# Autodesk Inventor assembly: BV-ASM-222-106
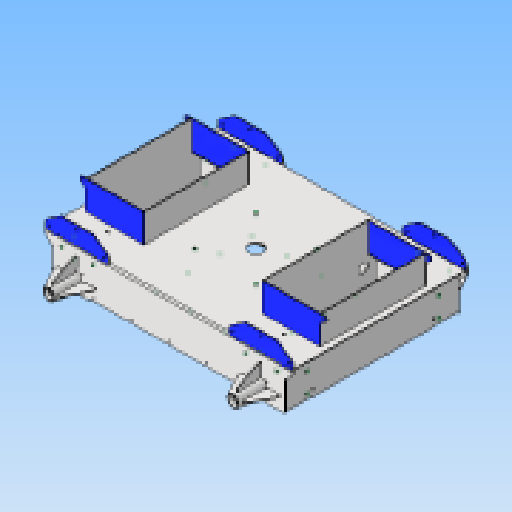
[picture p0: Inventor's stored thumbnail of the model, 512x512]
Saved by Autodesk Inventor 2025.4 (Build 294407000, 407)
## iProperties
Created: 2025-12-05
Part Number: BV-ASM-222-106
Document SubType Name: Assembly
Designer: josh
Mass: 150690 g
Surface Area: 81440.8 cm^2
Volume: 19196.2 cm^3
Density: 7.85 g/cm^3
Description: Base Weldment
Author: josh
## iProperties of the stored document MemberDocs/x54frrunuJ0si20qmEdadrqylTg
Created: 2025-12-05
Document SubType Name: Assembly
Designer: josh
Mass: 150690 g
Surface Area: 81440.8 cm^2
Volume: 19196.2 cm^3
Density: 7.85 g/cm^3
Author: josh
## iProperties of the stored document MemberDocs/xFojfi5agHc25u2sk4sonpsnbLc
Created: 2025-12-05
Document SubType Name: Assembly
Designer: josh
Mass: 150690 g
Surface Area: 81440.8 cm^2
Volume: 19196.2 cm^3
Density: 7.85 g/cm^3
Author: josh
## Documents named in this file (30)
- R:\A1- Neuweg Design Data\OM Robotics\BASE VEHICLE DESIGN PROJECT\BV-ASM-222-106.iam
- R:\A1- Neuweg Design Data\OM Robotics\BASE VEHICLE DESIGN PROJECT\BV-222-106.ipt
- R:\A1- Neuweg Design Data\OM Robotics\BASE VEHICLE DESIGN PROJECT\BV-222-107.ipt
- R:\A1- Neuweg Design Data\OM Robotics\BASE VEHICLE DESIGN PROJECT\BV-222-109.ipt
- R:\A1- Neuweg Design Data\OM Robotics\BASE VEHICLE DESIGN PROJECT\BV-222-116.ipt
- R:\A1- Neuweg Design Data\OM Robotics\BASE VEHICLE DESIGN PROJECT\BV-222-117.ipt
- R:\A1- Neuweg Design Data\OM Robotics\BASE VEHICLE DESIGN PROJECT\BV-222-118.ipt
- R:\A1- Neuweg Design Data\OM Robotics\BASE VEHICLE DESIGN PROJECT\BV-ASM-222-104.iam
- R:\A1- Neuweg Design Data\OM Robotics\BASE VEHICLE DESIGN PROJECT\BV-ASM-222-105.iam
- R:\A1- Neuweg Design Data\OM Robotics\BASE VEHICLE DESIGN PROJECT\BV-222-105.ipt
- R:\A1- Neuweg Design Data\OM Robotics\BASE VEHICLE DESIGN PROJECT\BV-222-108.ipt
- R:\A1- Neuweg Design Data\OM Robotics\BASE VEHICLE DESIGN PROJECT\BV-222-112.ipt
- R:\A1- Neuweg Design Data\OM Robotics\BASE VEHICLE DESIGN PROJECT\BV-222-119.ipt
- R:\A1- Neuweg Design Data\OM Robotics\BASE VEHICLE DESIGN PROJECT\BV-222-120.ipt
- R:\A1- Neuweg Design Data\OM Robotics\BASE VEHICLE DESIGN PROJECT\0222-110.ipt
- R:\A1- Neuweg Design Data\OM Robotics\BASE VEHICLE DESIGN PROJECT\3_8-16 x 5_8 Flange Bolt.ipt
- R:\A1- Neuweg Design Data\OM Robotics\BASE VEHICLE DESIGN PROJECT\1_4-20 UNC x 0.625.ipt
- R:\A1- Neuweg Design Data\OM Robotics\BASE VEHICLE DESIGN PROJECT\90128A277.ipt
- R:\A1- Neuweg Design Data\OM Robotics\BASE VEHICLE DESIGN PROJECT\91290A446.ipt
- R:\A1- Neuweg Design Data\OM Robotics\BASE VEHICLE DESIGN PROJECT\91259A177.ipt
- R:\A1- Neuweg Design Data\OM Robotics\BASE VEHICLE DESIGN PROJECT\94945A213.ipt
- R:\A1- Neuweg Design Data\OM Robotics\BASE VEHICLE DESIGN PROJECT\BV-ASM-222-102.iam
- R:\A1- Neuweg Design Data\OM Robotics\BASE VEHICLE DESIGN PROJECT\30205.ipt
- R:\A1- Neuweg Design Data\OM Robotics\BASE VEHICLE DESIGN PROJECT\251105 Motor_Drive.ipt
- R:\A1- Neuweg Design Data\OM Robotics\BASE VEHICLE DESIGN PROJECT\22x10x8.ipt
- R:\A1- Neuweg Design Data\OM Robotics\BASE VEHICLE DESIGN PROJECT\0222-113-2.ipt
- R:\A1- Neuweg Design Data\OM Robotics\BASE VEHICLE DESIGN PROJECT\97260A109.ipt
- R:\A1- Neuweg Design Data\OM Robotics\BASE VEHICLE DESIGN PROJECT\93560A112.ipt
- R:\A1- Neuweg Design Data\OM Robotics\BASE VEHICLE DESIGN PROJECT\1199N323.ipt
- R:\A1- Neuweg Design Data\OM Robotics\BASE VEHICLE DESIGN PROJECT\BV-ASM-222-103.iam
## Components (30 placed, 8 different names)
1. BV-ASM-222-104:1 [sub-assembly] — Flush:11, Flush:12, Flush:13
2. BV-ASM-222-105:1 [sub-assembly]
3. BV-222-106:1
4. BV-222-107:1
5. BV-222-109:1
6. BV-222-116:1
7. BV-222-118:1
8. BV-222-106:2
9. BV-222-107:2
10. BV-222-109:2
11. BV-222-116:2
12. BV-222-118:2
13. BV-222-109:3
14. BV-222-116:3
15. BV-222-118:3
16. BV-222-109:4
17. BV-222-116:4
18. BV-222-118:4
19. BV-222-117:1
20. BV-222-117:2
21. BV-222-117:3
22. BV-222-117:4
23. BV-222-117:5
24. BV-222-117:6
25. BV-222-117:7
26. BV-222-117:9
27. BV-222-117:10
28. BV-222-117:8
29. BV-222-117:11
30. BV-222-117:12
## Component patterns: (3 elements, first: BV-222-117:1), (3 elements, first: BV-222-117:4), (3 elements, first: BV-222-117:7), (3 elements, first: BV-222-117:8)
## Relationships (3: Flush 3)
- Flush:11: BV-ASM-222-104:1
- Flush:12: BV-ASM-222-104:1
- Flush:13: BV-ASM-222-104:1
